# Autodesk Inventor assembly: DaVinci head and guide assy
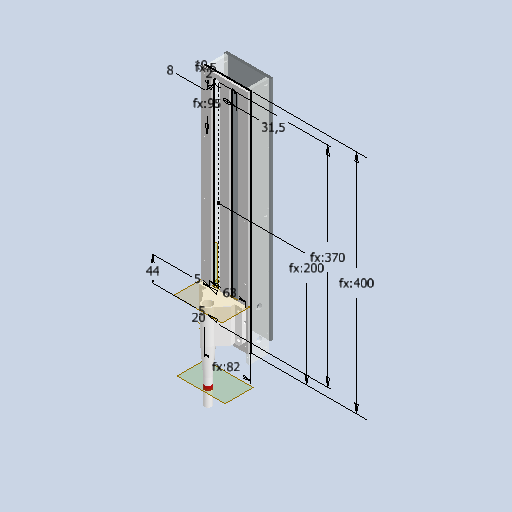
[picture p0: Inventor's stored thumbnail of the model, 512x512]
Saved by Autodesk Inventor 2022 (Build 260153000, 153)
## iProperties
Created: 2021-11-04
Part Number: DaVinci head and guide assy
Document SubType Name: Assembly
Designer: espen
Mass: 587.663 g
Surface Area: 2187.27 cm^2
Volume: 519.448 cm^3
Density: 1.13132 g/cm^3
Author: espen
## Documents named in this file (5)
- C:\Users\alexw\Documents\Inventor\Projects\03_CurrentProjects\MasterThesis\PSM_V1_Rillenkugellager\DaVinci head and guide assy.iam
- C:\Users\alexw\Documents\Inventor\Projects\03_CurrentProjects\MasterThesis\PSM_V1_Rillenkugellager\Slot profile.ipt
- C:\Users\alexw\Documents\Inventor\Projects\03_CurrentProjects\MasterThesis\PSM_V1_Rillenkugellager\Side plate profile.ipt
- C:\Users\alexw\Documents\Inventor\Projects\03_CurrentProjects\MasterThesis\PSM_V1_Rillenkugellager\Back plate profile.ipt
- C:\Users\alexw\Documents\Inventor\Projects\03_CurrentProjects\MasterThesis\PSM_V1_Rillenkugellager\Guide.ipt
## Components (5 placed, 4 different names)
1. Slot profile:1 — Mate:1, Flush:1, Flush:2, Mate:2, Mate:3, Mate:5, Mate:6, Mate:11, Mate:12, Mate:13
2. Side plate profile:1 — Mate:2, Mate:3, Mate:8, Mate:9, Passend:14, Passend:15, Winkel:1, Winkel:2
3. Side plate profile:2 — Mate:5, Mate:6
4. Back plate profile:1 — Mate:8, Mate:9
5. Guide:1 — Mate:11, Mate:12, Mate:13
## Relationships (21: Mate 16, Flush 2, Angle 2, Symmetry 1)
- Mate:1: Slot profile:1
- Flush:1: Slot profile:1
- Flush:2: Slot profile:1
- Mate:2: Slot profile:1 ↔ Side plate profile:1
- Mate:3: Slot profile:1 ↔ Side plate profile:1
- Mate:5: Slot profile:1 ↔ Side plate profile:2
- Mate:6: Slot profile:1 ↔ Side plate profile:2
- Mate:8: Side plate profile:1 ↔ Back plate profile:1
- Mate:9: Side plate profile:1 ↔ Back plate profile:1
- Mate:11: Slot profile:1 ↔ Guide:1
- Mate:12: Slot profile:1 ↔ Guide:1
- Mate:13: Slot profile:1 ↔ Guide:1
- Passend:14 [Mate]: Side plate profile:1
- Passend:15 [Mate]: Side plate profile:1
- Passend:16 [Mate]
- Winkel:1 [Angle] (0 deg): Side plate profile:1
- Passend:17 [Mate]
- Winkel:2 [Angle] (0 deg): Side plate profile:1
- Symmetrie:1
- Passend:18 [Mate]
- Passend:19 [Mate]
